# Autodesk Inventor assembly: assembily_v2
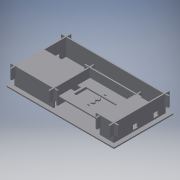
[picture p0: Inventor's stored thumbnail of the model, 180x180]
Saved by Autodesk Inventor 2017.2 (Build 212233000, 233)
## iProperties
Created: 2017-06-09
Part Number: assembily_v2
Document SubType Name: Assembly
Designer: SandeepSH
Author: SandeepSH
## Documents named in this file (12)
- C:\Users\SandeepSH\Dropbox\MSC\Project\inventor\lcv1\assembily_v2.iam
- C:\Users\SandeepSH\Dropbox\MSC\Project\inventor\lcv1\base_v2.ipt
- C:\Users\SandeepSH\Dropbox\MSC\Project\inventor\lcv1\cham_right_v2.ipt
- C:\Users\SandeepSH\Dropbox\MSC\Project\inventor\lcv1\cham_left_v2.ipt
- C:\Users\SandeepSH\Dropbox\MSC\Project\inventor\lcv1\cham_back_v2.ipt
- C:\Users\SandeepSH\Dropbox\MSC\Project\inventor\lcv1\front_left_v2.ipt
- C:\Users\SandeepSH\Dropbox\MSC\Project\inventor\lcv1\front_right_v2.ipt
- C:\Users\SandeepSH\Dropbox\MSC\Project\inventor\lcv1\side_v2.ipt
- C:\Users\SandeepSH\Dropbox\MSC\Project\inventor\lcv1\top_left_v2.ipt
- C:\Users\SandeepSH\Dropbox\MSC\Project\inventor\lcv1\top_right_v2.ipt
- C:\Users\SandeepSH\Dropbox\MSC\Project\inventor\lcv1\back_v2.ipt
- C:\Users\SandeepSH\Dropbox\MSC\Project\inventor\lcv1\roof_v2.ipt
## Components (12 placed, 11 different names)
1. base_v2:1 — Mate:1, Mate:2, Mate:5, Mate:6, Mate:9, Mate:10, Mate:12, Mate:13, Mate:16, Mate:17, Mate:18, Mate:19, Mate:20, Mate:21, Mate:22, Mate:27, Mate:28
2. cham_right_v2:1 — Mate:1, Mate:2
3. cham_back_v2:1 — Mate:5, Mate:6
4. front_right_v2:1 — Mate:9, Mate:10
5. side_v2:2 — Mate:12, Mate:13, Mate:16, Mate:25, Mate:26
6. cham_left_v2:1 — Mate:17, Mate:18
7. front_left_v2:1 — Mate:19, Mate:20, Mate:23, Mate:24
8. side_v2:3 — Mate:21, Mate:22
9. top_left_v2:1 — Mate:23, Mate:24
10. top_right_v2:1 — Mate:25, Mate:26
11. back_v2:1 — Mate:27, Mate:28
12. roof_v2:1
## Relationships (21: Mate 21)
- Mate:1: base_v2:1 ↔ cham_right_v2:1
- Mate:2: base_v2:1 ↔ cham_right_v2:1
- Mate:5: base_v2:1 ↔ cham_back_v2:1
- Mate:6: base_v2:1 ↔ cham_back_v2:1
- Mate:9: base_v2:1 ↔ front_right_v2:1
- Mate:10: base_v2:1 ↔ front_right_v2:1
- Mate:12: base_v2:1 ↔ side_v2:2
- Mate:13: base_v2:1 ↔ side_v2:2
- Mate:16: base_v2:1 ↔ side_v2:2
- Mate:17: base_v2:1 ↔ cham_left_v2:1
- Mate:18: base_v2:1 ↔ cham_left_v2:1
- Mate:19: base_v2:1 ↔ front_left_v2:1
- Mate:20: base_v2:1 ↔ front_left_v2:1
- Mate:21: base_v2:1 ↔ side_v2:3
- Mate:22: base_v2:1 ↔ side_v2:3
- Mate:23: front_left_v2:1 ↔ top_left_v2:1
- Mate:24: front_left_v2:1 ↔ top_left_v2:1
- Mate:25: side_v2:2 ↔ top_right_v2:1
- Mate:26: side_v2:2 ↔ top_right_v2:1
- Mate:27: base_v2:1 ↔ back_v2:1
- Mate:28: base_v2:1 ↔ back_v2:1
